# Autodesk Inventor assembly: Contraction Assembly
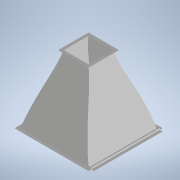
[picture p0: Inventor's stored thumbnail of the model, 180x180]
Saved by Autodesk Inventor 2022 (Build 260153000, 153)
## iProperties
Created: 2022-03-06
Part Number: Contraction Assembly
Document SubType Name: Assembly
Designer: calvi
Author: calvi
## Documents named in this file (3)
- E:\Dr. A Muchiri\Wind tunnel_Dr.A Muchiri\Contraction Assembly.iam
- E:\Dr. A Muchiri\Wind tunnel_Dr.A Muchiri\Contraction.ipt
- E:\Dr. A Muchiri\Wind tunnel_Dr.A Muchiri\Fastening Frame.ipt
## Components (2 placed, 2 different names)
1. Contraction:1 — Mate:1, Flush:1, Flush:2
2. Fastening Frame:1 — Mate:1, Flush:1, Flush:2
## Relationships (3: Flush 2, Mate 1)
- Mate:1: Contraction:1 ↔ Fastening Frame:1
- Flush:1: Contraction:1 ↔ Fastening Frame:1
- Flush:2: Contraction:1 ↔ Fastening Frame:1
